# Autodesk Inventor assembly: D-050.50 Capacitive Sensors
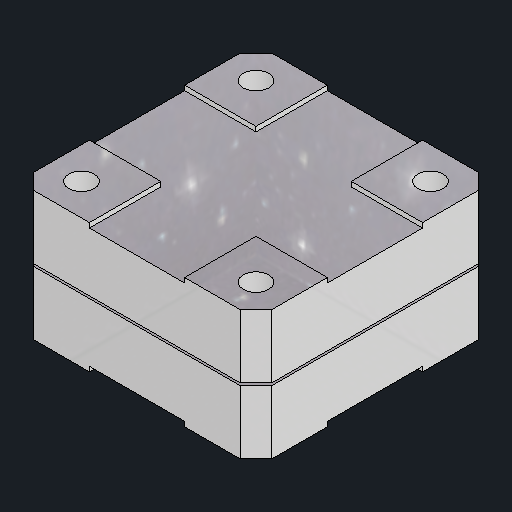
[picture p0: Inventor's stored thumbnail of the model, 512x512]
Saved by Autodesk Inventor 2025.2 (Build 292293000, 293)
## iProperties
Created: 2025-04-13
Part Number: D-050.50 Capacitive Sensors
Document SubType Name: Assembly
Designer: Kacper Mik
Mass: 4.165 g
Surface Area: 15.7584 cm^2
Volume: 1.54259 cm^3
Density: 2.7 g/cm^3
Author: Kacper Mik
## Documents named in this file (2)
- C:\Users\kacpe\Documents\STUDIA\INŻYNIERKA\Nanotwardościomierz\Nanotwardosciomierz inventor\zesp_czujnikow.iam
- C:\Users\kacpe\Documents\STUDIA\INŻYNIERKA\Nanotwardościomierz\Nanotwardosciomierz inventor\D-100.00 Capacitive Sensor.ipt
## Components (2 placed, 1 different names)
1. D-100.00 Capacitive Sensor:1 — Angle:1, Angle:3, Mate:1, Angle:5, Mate:2
2. D-100.00 Capacitive Sensor:2 — Mate:1, Angle:4, Angle:5, Mate:2
## Relationships (6: Angle 4, Mate 2)
- Angle:1 (0 deg): D-100.00 Capacitive Sensor:1
- Angle:3 (0 deg): D-100.00 Capacitive Sensor:1
- Mate:1 (0.15 mm): D-100.00 Capacitive Sensor:1 ↔ D-100.00 Capacitive Sensor:2
- Angle:4 (0 deg): D-100.00 Capacitive Sensor:2
- Angle:5 (0 deg): D-100.00 Capacitive Sensor:1 ↔ D-100.00 Capacitive Sensor:2
- Mate:2: D-100.00 Capacitive Sensor:1 ↔ D-100.00 Capacitive Sensor:2
